# Autodesk Inventor assembly: 25
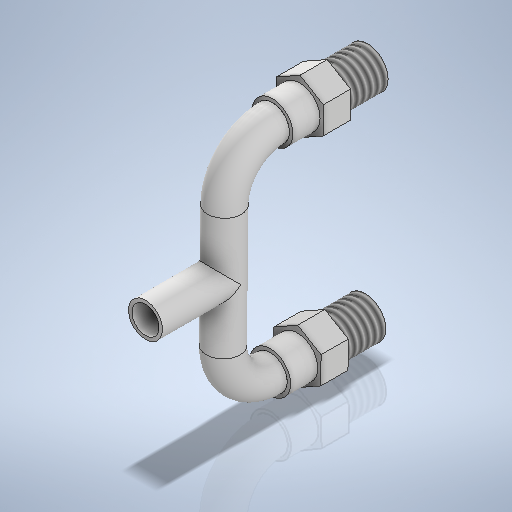
[picture p0: Inventor's stored thumbnail of the model, 512x512]
Saved by Autodesk Inventor 2025.1 (Build 291241000, 241)
## iProperties
Created: 2024-09-13
Part Number: 25
Document SubType Name: Assembly
Designer: ffogue
Author: ffogue
## Documents named in this file (3)
- C:\Users\ffogue\Documents\Inventor\Single cylinder Steam Engine\25.iam
- C:\Users\ffogue\Documents\Inventor\Single cylinder Steam Engine\25.ipt
- C:\Users\ffogue\Documents\Inventor\Single cylinder Steam Engine\25.1.ipt
## Components (3 placed, 2 different names)
1. 25:1 — Mate:1, Cylindrical:1, Mate:3, Cylindrical:2
2. 25.1:1 — Mate:2, Cylindrical:1
3. 25.1:2 — Mate:4, Cylindrical:2
## Relationships (6: Mate 4, CylindricalJoint 2)
- Mate:1: 25:1
- Mate:2: 25.1:1
- Cylindrical:1: 25:1 ↔ 25.1:1
- Mate:3: 25:1
- Mate:4: 25.1:2
- Cylindrical:2: 25:1 ↔ 25.1:2
